# Autodesk Inventor assembly: triangulo con anclajes
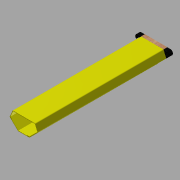
[picture p0: Inventor's stored thumbnail of the model, 180x180]
Saved by Autodesk Inventor 2014 (Build 180170000, 170)
## iProperties
Created: 2016-10-24
Part Number: triangulo con anclajes
Document SubType Name: Assembly
Designer: Cristian
Author: Cristian
## Documents named in this file (6)
- C:\Users\Cristian\Desktop\ANTENA MESH\triangulo con anclajes.iam
- C:\Users\Cristian\Desktop\ANTENA MESH\triangulo madera 2.ipt
- C:\Users\Cristian\Desktop\ANTENA MESH\fijaciones triangulo p1.ipt
- C:\Users\Cristian\Desktop\ANTENA MESH\fijaciones triangulo p2.ipt
- C:\Users\Cristian\Desktop\ANTENA MESH\fijaciones triangulo p3.ipt
- C:\Users\Cristian\Desktop\piezas 3d hechas y por hacer\soportes porta pliegos\aluco de metro.ipt
## Components (5 placed, 5 different names)
1. triangulo madera 2:1 — Mate:1, Mate:2, Mate:3, Mate:4, Flush:1, Mate:5, Flush:2, Mate:6, Mate:7, Flush:3, Mate:8, Mate:9, Flush:4, Flush:5
2. fijaciones triangulo p2:1 — Mate:4, Flush:1, Mate:5
3. fijaciones triangulo p3:1 — Flush:2, Mate:6, Mate:7
4. fijaciones triangulo p1:1 — Flush:3, Mate:8, Mate:9
5. aluco de metro:1 — Flush:4, Flush:5
## Relationships (14: Mate 9, Flush 5)
- Mate:1: triangulo madera 2:1
- Mate:2: triangulo madera 2:1
- Mate:3: triangulo madera 2:1
- Mate:4: triangulo madera 2:1 ↔ fijaciones triangulo p2:1
- Flush:1: triangulo madera 2:1 ↔ fijaciones triangulo p2:1
- Mate:5: triangulo madera 2:1 ↔ fijaciones triangulo p2:1
- Flush:2: triangulo madera 2:1 ↔ fijaciones triangulo p3:1
- Mate:6: triangulo madera 2:1 ↔ fijaciones triangulo p3:1
- Mate:7: triangulo madera 2:1 ↔ fijaciones triangulo p3:1
- Flush:3: triangulo madera 2:1 ↔ fijaciones triangulo p1:1
- Mate:8: triangulo madera 2:1 ↔ fijaciones triangulo p1:1
- Mate:9: triangulo madera 2:1 ↔ fijaciones triangulo p1:1
- Flush:4: triangulo madera 2:1 ↔ aluco de metro:1
- Flush:5: triangulo madera 2:1 ↔ aluco de metro:1
